# Autodesk Inventor assembly: Planktoscope_Mini_Electronicbase
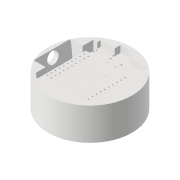
[picture p0: Inventor's stored thumbnail of the model, 180x180]
Saved by Autodesk Inventor 2022 (Build 260153000, 153)
## iProperties
Created: 2022-12-07
Part Number: Planktoscope_Mini_Electronicbase
Document SubType Name: Assembly
Designer: diederichbenedict
Author: diederichbenedict
## Documents named in this file (4)
- C:\Users\diederichbenedict\Dropbox\Dokumente\Promotion\PROJECTS\Matchboxscope\INVENTOR\MATCHBOXSCOPE\Planktoscope_Mini_Electronicbase.iam
- C:\Users\diederichbenedict\Dropbox\Dokumente\Promotion\PROJECTS\Matchboxscope\INVENTOR\MATCHBOXSCOPE\Planktoscope_Mini_Electronicbase.ipt
- C:\Users\diederichbenedict\Dropbox\Dokumente\Promotion\PROJECTS\Matchboxscope\INVENTOR\MATCHBOXSCOPE\00_Wemos-Mini-D1-ESP32.ipt
- C:\Users\diederichbenedict\Dropbox\Dokumente\Promotion\PROJECTS\Matchboxscope\INVENTOR\MATCHBOXSCOPE\00_ULN2003 Stepper Driver.ipt
## Components (3 placed, 3 different names)
1. 00_ULN2003 Stepper Driver:1
2. 00_Wemos-Mini-D1-ESP32:1
3. Planktoscope_Mini_Electronicbase:1
## Relationships (1: Mate 1)
- [Mate] (12 mm): 00_ULN2003 Stepper Driver:1 ↔ 00_Wemos-Mini-D1-ESP32:1
